# Autodesk Inventor assembly: ring
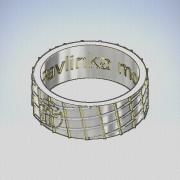
[picture p0: Inventor's stored thumbnail of the model, 180x180]
Saved by Autodesk Inventor 2018 (Build 220112000, 112)
## iProperties
Created: 2019-09-11
Part Number: ring
Document SubType Name: Assembly
Designer: dsikar
Author: dsikar
## Documents named in this file (5)
- C:\Users\dsikar\Documents\Inventor\volleyball-ring\assemblies\ring.iam
- C:\Users\dsikar\Documents\Inventor\volleyball-ring\parts\net.ipt
- C:\Users\dsikar\Documents\Inventor\volleyball-ring\parts\net2-hozontal.ipt
- C:\Users\dsikar\Documents\Inventor\volleyball-ring\parts\ball.ipt
- C:\Users\dsikar\Documents\Inventor\volleyball-ring\parts\inside-text.ipt
## Components (4 placed, 4 different names)
1. net:1 — Mate:1, Mate:2, Mate:4, Mate:9
2. net2-hozontal:1 — Mate:3
3. ball:1 — Mate:6, Mate:7
4. inside-text:1 — Mate:8, Mate:9
## Relationships (8: Mate 8)
- Mate:1: net:1
- Mate:2: net:1
- Mate:3: net2-hozontal:1
- Mate:4: net:1
- Mate:6: ball:1
- Mate:7: ball:1
- Mate:8: inside-text:1
- Mate:9: net:1 ↔ inside-text:1
